# Autodesk Inventor assembly: case_roboclaw_assembly
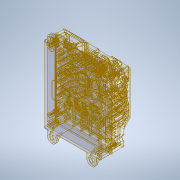
[picture p0: Inventor's stored thumbnail of the model, 180x180]
Saved by Autodesk Inventor 2020 (Build 240168000, 168)
## iProperties
Created: 2019-11-08
Part Number: case_roboclaw_assembly
Document SubType Name: Assembly
Designer: maste
Author: maste
## Documents named in this file (3)
- C:\Users\maste\Documents\GitHub\autobot\robot_model\case_roboclaw_assembly.iam
- C:\Users\maste\Documents\GitHub\autobot\robot_model\roboclaw_case\ROBOCLAW_CASE_15A_30A_45A.ipt
- C:\Users\maste\Documents\GitHub\autobot\robot_model\roboclaw_2x15A\MC15A_V5.iam
## Components (2 placed, 2 different names)
1. ROBOCLAW_CASE_15A_30A_45A:1 — Mate:1, Mate:2, Mate:3
2. MC15A_V5:1 [sub-assembly] — Mate:1, Mate:2, Mate:3
## Relationships (3: Mate 3)
- Mate:1: ROBOCLAW_CASE_15A_30A_45A:1 ↔ MC15A_V5:1
- Mate:2: ROBOCLAW_CASE_15A_30A_45A:1 ↔ MC15A_V5:1
- Mate:3: ROBOCLAW_CASE_15A_30A_45A:1 ↔ MC15A_V5:1
